# Autodesk Inventor assembly: robot
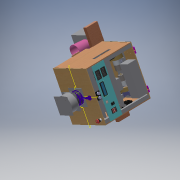
[picture p0: Inventor's stored thumbnail of the model, 180x180]
Saved by Autodesk Inventor 2019 (Build 230136000, 136)
## iProperties
Created: 2020-02-15
Part Number: robot
Document SubType Name: Assembly
Designer: franc
Author: franc
## Documents named in this file (20)
- C:\Users\franc\Desktop\EsialRobotik\Mecanique\2020\robot\robot.iam
- C:\Users\franc\Desktop\EsialRobotik\Mecanique\base_roulante\baseRoulante.iam
- C:\Users\franc\Desktop\EsialRobotik\Mecanique\2020\robot\socle-robot.ipt
- C:\Users\franc\Desktop\EsialRobotik\Mecanique\composants\Profile\calle.iam
- C:\Users\franc\Desktop\EsialRobotik\Mecanique\composants\Profile\equerreEtage.ipt
- C:\Users\franc\Desktop\EsialRobotik\Mecanique\2020\robot\profile_alu.ipt
- C:\Users\franc\Desktop\EsialRobotik\Mecanique\2020\robot\cote.ipt
- C:\Users\franc\Desktop\EsialRobotik\Mecanique\2020\robot\support-pinces.ipt
- C:\Users\franc\Desktop\EsialRobotik\Mecanique\2020\robot\pince a linge.ipt
- C:\Users\franc\Desktop\EsialRobotik\Mecanique\composants\Batterie\grosse-batterie.ipt
- C:\Users\franc\Desktop\EsialRobotik\Mecanique\composants\Batterie\petite-batterie.ipt
- C:\Users\franc\Desktop\EsialRobotik\Mecanique\2020\elements\ecueil-complet.iam
- C:\Users\franc\Desktop\EsialRobotik\Mecanique\2020\robot\étage.ipt
- C:\Users\franc\Desktop\EsialRobotik\Mecanique\2020\robot\support_arriere.iam
- C:\Users\franc\Desktop\EsialRobotik\Mecanique\2020\robot\toit.iam
- C:\Users\franc\Desktop\EsialRobotik\Mecanique\composants\AX12\AX12.iam
- C:\Users\franc\Desktop\EsialRobotik\Mecanique\composants\AX12\F3.ipt
- C:\Users\franc\Desktop\EsialRobotik\Mecanique\2020\robot\bras-manche.ipt
- C:\Users\franc\Desktop\EsialRobotik\Mecanique\2020\elements\bordure.ipt
- C:\Users\franc\Desktop\EsialRobotik\Mecanique\composants\SRF04\SRF04_sur_support.iam
## Components (48 placed, 19 different names)
1. baseRoulante:1 [sub-assembly] — Placage:1, Placage:2, Placage:3
2. socle-robot:1 — Placage:1, Placage:2, Placage:3, Placage:4, Placage:5, Placage:6, Placage:7, Placage:8, Placage:9, Placage:10, Placage:11, Placage:12, Placage:13, Placage:14, Placage:15, Placage:16, Placage:17, Placage:18, Placage:19, Placage:20, Placage:21, Placage:22, Placage:23, Placage:24, Placage:25, Placage:26, Placage:27, Placage:28, Placage:30, Placage:32, Placage:33, Placage:37, Placage:39, Placage:52, Affleurement:8, Placage:58, Placage:85
3. calle:1 [sub-assembly] — Placage:7, Placage:8, Placage:9
4. calle:2 [sub-assembly] — Placage:6, Placage:10, Placage:11
5. calle:3 [sub-assembly] — Placage:4, Placage:12, Placage:13
6. calle:4 [sub-assembly] — Placage:5, Placage:14, Placage:15, Affleurement:21
7. equerreEtage:1 — Placage:16, Placage:22, Placage:23, Placage:35, Affleurement:4
8. equerreEtage:2 — Placage:17, Placage:24, Placage:25, Placage:31, Affleurement:2
9. equerreEtage:3 — Placage:18, Placage:26, Placage:27, Placage:29, Affleurement:1
10. equerreEtage:4 — Placage:19, Placage:20, Placage:21, Placage:34, Affleurement:3
11. profile_alu:1 — Placage:28, Placage:29, Affleurement:1, Placage:59, Placage:70, Placage:74
12. profile_alu:2 — Placage:32, Placage:34, Affleurement:3, Affleurement:10, Placage:54, Placage:56, Placage:72, Placage:76, Placage:89, Affleurement:14, Placage:101, Placage:115
13. profile_alu:3 — Placage:33, Placage:35, Affleurement:4, Affleurement:5, Placage:78, Placage:82, Placage:88, Affleurement:13, Placage:107
14. profile_alu:4 — Placage:30, Placage:31, Affleurement:2, Placage:36, Placage:80, Placage:84
15. cote:1 — Placage:36, Placage:37, Affleurement:5, Affleurement:11, Placage:77, Placage:79, Placage:81, Placage:83, Placage:106
16. cote:2 — Placage:39, Affleurement:10, Placage:54, Placage:55, Placage:57, Placage:60, Placage:69, Placage:71, Placage:73, Placage:75, Placage:90, Affleurement:15, Affleurement:16, Placage:100, Placage:117, Placage:119, Affleurement:22
17. support-pinces:1 — Placage:41, Placage:42, Placage:43, Placage:44, Placage:45, Placage:47, Placage:48, Placage:49, Placage:50, Placage:51, Angle:1, Angle:2, Angle:3, Angle:4, Angle:5, Placage:55, Affleurement:11, Affleurement:22
18. pince a linge:1 — Placage:41, Placage:47, Angle:1
19. pince a linge:2 — Placage:42, Placage:48, Angle:2
20. pince a linge:3 — Placage:43, Placage:49, Angle:3
21. pince a linge:4 — Placage:44, Placage:50, Angle:4
22. pince a linge:5 — Placage:45, Placage:51, Angle:5
23. grosse-batterie:1 — Placage:52, Affleurement:8, Placage:115
24. petite-batterie:1 — Placage:116, Affleurement:18, Placage:117
25. ecueil-complet:1 [sub-assembly] — Placage:118, Affleurement:19, Affleurement:20, Placage:120
26. étage:1 — Placage:56, Placage:57, Placage:58, Placage:61, Placage:62, Placage:63, Placage:64, Placage:99, Placage:105, Placage:116, Affleurement:18
27. étage:2 — Placage:59, Placage:60, Placage:65, Placage:66, Placage:67, Placage:68, Placage:85
28. equerreEtage:5 — Placage:64, Placage:83, Placage:84
29. equerreEtage:6 — Placage:63, Placage:81, Placage:82
30. equerreEtage:7 — Placage:61, Placage:69, Placage:70
31. equerreEtage:8 — Placage:62, Placage:71, Placage:72
32. equerreEtage:9 — Placage:68, Placage:77, Placage:78
33. equerreEtage:10 — Placage:65, Placage:73, Placage:74
34. equerreEtage:11 — Placage:67, Placage:79, Placage:80
35. equerreEtage:12 — Placage:66, Placage:75, Placage:76
36. support_arriere:1 [sub-assembly] — Placage:88, Placage:89, Affleurement:13, Affleurement:14
37. toit:1 [sub-assembly] — Placage:90, Affleurement:15, Affleurement:16, Placage:120, Placage:121, Placage:122, Placage:123, Placage:124, Placage:125, Placage:126, Placage:127, Placage:128
38. AX12:1 [sub-assembly] — Placage:96, Placage:97, Placage:98, Placage:100, Placage:111, Placage:112, Placage:113
39. AX12:2 [sub-assembly] — Placage:102, Placage:103, Placage:104, Placage:106, Placage:108, Placage:109, Placage:110
40. F3:1 — Placage:96, Placage:97, Placage:98, Placage:99, Placage:101
41. F3:2 — Placage:102, Placage:103, Placage:104, Placage:105, Placage:107
42. bras-manche:1 — Placage:108, Placage:109, Placage:110
43. bras-manche:2 — Placage:111, Placage:112, Placage:113
44. bordure:1 — Placage:118, Affleurement:19, Affleurement:20, Affleurement:21, Placage:119
45. SRF04_sur_support:1 [sub-assembly] — Placage:125, Placage:126
46. SRF04_sur_support:2 [sub-assembly] — Placage:127, Placage:128
47. SRF04_sur_support:3 [sub-assembly] — Placage:121, Placage:122
48. SRF04_sur_support:4 [sub-assembly] — Placage:123, Placage:124
## Relationships (138: Mate 116, Flush 17, Angle 5)
- Placage:1 [Mate]: baseRoulante:1 ↔ socle-robot:1
- Placage:2 [Mate]: baseRoulante:1 ↔ socle-robot:1
- Placage:3 [Mate]: baseRoulante:1 ↔ socle-robot:1
- Placage:4 [Mate]: socle-robot:1 ↔ calle:3
- Placage:5 [Mate]: socle-robot:1 ↔ calle:4
- Placage:6 [Mate]: socle-robot:1 ↔ calle:2
- Placage:7 [Mate]: socle-robot:1 ↔ calle:1
- Placage:8 [Mate]: socle-robot:1 ↔ calle:1
- Placage:9 [Mate]: socle-robot:1 ↔ calle:1
- Placage:10 [Mate]: socle-robot:1 ↔ calle:2
- Placage:11 [Mate]: socle-robot:1 ↔ calle:2
- Placage:12 [Mate]: socle-robot:1 ↔ calle:3
- Placage:13 [Mate]: socle-robot:1 ↔ calle:3
- Placage:14 [Mate]: socle-robot:1 ↔ calle:4
- Placage:15 [Mate]: socle-robot:1 ↔ calle:4
- Placage:16 [Mate]: socle-robot:1 ↔ equerreEtage:1
- Placage:17 [Mate]: socle-robot:1 ↔ equerreEtage:2
- Placage:18 [Mate]: socle-robot:1 ↔ equerreEtage:3
- Placage:19 [Mate]: socle-robot:1 ↔ equerreEtage:4
- Placage:20 [Mate]: socle-robot:1 ↔ equerreEtage:4
- Placage:21 [Mate]: socle-robot:1 ↔ equerreEtage:4
- Placage:22 [Mate]: socle-robot:1 ↔ equerreEtage:1
- Placage:23 [Mate]: socle-robot:1 ↔ equerreEtage:1
- Placage:24 [Mate]: socle-robot:1 ↔ equerreEtage:2
- Placage:25 [Mate]: socle-robot:1 ↔ equerreEtage:2
- Placage:26 [Mate]: socle-robot:1 ↔ equerreEtage:3
- Placage:27 [Mate]: socle-robot:1 ↔ equerreEtage:3
- Placage:28 [Mate]: socle-robot:1 ↔ profile_alu:1
- Placage:29 [Mate]: equerreEtage:3 ↔ profile_alu:1
- Affleurement:1 [Flush]: equerreEtage:3 ↔ profile_alu:1
- Placage:30 [Mate]: socle-robot:1 ↔ profile_alu:4
- Placage:31 [Mate]: equerreEtage:2 ↔ profile_alu:4
- Affleurement:2 [Flush]: equerreEtage:2 ↔ profile_alu:4
- Placage:32 [Mate]: socle-robot:1 ↔ profile_alu:2
- Placage:33 [Mate]: socle-robot:1 ↔ profile_alu:3
- Placage:34 [Mate]: equerreEtage:4 ↔ profile_alu:2
- Affleurement:3 [Flush]: equerreEtage:4 ↔ profile_alu:2
- Placage:35 [Mate]: equerreEtage:1 ↔ profile_alu:3
- Affleurement:4 [Flush]: equerreEtage:1 ↔ profile_alu:3
- Placage:36 [Mate]: profile_alu:4 ↔ cote:1
- Placage:37 [Mate]: socle-robot:1 ↔ cote:1
- Affleurement:5 [Flush]: profile_alu:3 ↔ cote:1
- Placage:39 [Mate]: socle-robot:1 ↔ cote:2
- Placage:41 [Mate]: support-pinces:1 ↔ pince a linge:1
- Placage:42 [Mate]: support-pinces:1 ↔ pince a linge:2
- Placage:43 [Mate]: support-pinces:1 ↔ pince a linge:3
- Placage:44 [Mate]: support-pinces:1 ↔ pince a linge:4
- Placage:45 [Mate]: support-pinces:1 ↔ pince a linge:5
- Placage:47 [Mate]: support-pinces:1 ↔ pince a linge:1
- Placage:48 [Mate]: support-pinces:1 ↔ pince a linge:2
- Placage:49 [Mate]: support-pinces:1 ↔ pince a linge:3
- Placage:50 [Mate]: support-pinces:1 ↔ pince a linge:4
- Placage:51 [Mate]: support-pinces:1 ↔ pince a linge:5
- Angle:1 (0 deg): support-pinces:1 ↔ pince a linge:1
- Angle:2 (0 deg): support-pinces:1 ↔ pince a linge:2
- Angle:3 (0 deg): support-pinces:1 ↔ pince a linge:3
- Angle:4 (0 deg): support-pinces:1 ↔ pince a linge:4
- Angle:5 (0 deg): support-pinces:1 ↔ pince a linge:5
- Placage:52 [Mate]: socle-robot:1 ↔ grosse-batterie:1
- Affleurement:8 [Flush]: socle-robot:1 ↔ grosse-batterie:1
- Affleurement:10 [Flush]: profile_alu:2 ↔ cote:2
- Placage:54 [Mate]: profile_alu:2 ↔ cote:2
- Placage:55 [Mate]: cote:2 ↔ support-pinces:1
- Affleurement:11 [Flush] (-5 mm): cote:1 ↔ support-pinces:1
- Placage:56 [Mate]: profile_alu:2 ↔ étage:1
- Placage:57 [Mate]: cote:2 ↔ étage:1
- Placage:58 [Mate] (140 mm): socle-robot:1 ↔ étage:1
- Placage:59 [Mate]: profile_alu:1 ↔ étage:2
- Placage:60 [Mate]: cote:2 ↔ étage:2
- Placage:61 [Mate]: étage:1 ↔ equerreEtage:7
- Placage:62 [Mate]: étage:1 ↔ equerreEtage:8
- Placage:63 [Mate]: étage:1 ↔ equerreEtage:6
- Placage:64 [Mate]: étage:1 ↔ equerreEtage:5
- Placage:65 [Mate]: étage:2 ↔ equerreEtage:10
- Placage:66 [Mate]: étage:2 ↔ equerreEtage:12
- Placage:67 [Mate]: étage:2 ↔ equerreEtage:11
- Placage:68 [Mate]: étage:2 ↔ equerreEtage:9
- Placage:69 [Mate]: cote:2 ↔ equerreEtage:7
- Placage:70 [Mate]: profile_alu:1 ↔ equerreEtage:7
- Placage:71 [Mate]: cote:2 ↔ equerreEtage:8
- Placage:72 [Mate]: profile_alu:2 ↔ equerreEtage:8
- Placage:73 [Mate]: cote:2 ↔ equerreEtage:10
- Placage:74 [Mate]: profile_alu:1 ↔ equerreEtage:10
- Placage:75 [Mate]: cote:2 ↔ equerreEtage:12
- Placage:76 [Mate]: profile_alu:2 ↔ equerreEtage:12
- Placage:77 [Mate]: cote:1 ↔ equerreEtage:9
- Placage:78 [Mate]: profile_alu:3 ↔ equerreEtage:9
- Placage:79 [Mate]: cote:1 ↔ equerreEtage:11
- Placage:80 [Mate]: profile_alu:4 ↔ equerreEtage:11
- Placage:81 [Mate]: cote:1 ↔ equerreEtage:6
- Placage:82 [Mate]: profile_alu:3 ↔ equerreEtage:6
- Placage:83 [Mate]: cote:1 ↔ equerreEtage:5
- Placage:84 [Mate]: profile_alu:4 ↔ equerreEtage:5
- Placage:85 [Mate] (230 mm): socle-robot:1 ↔ étage:2
- Placage:88 [Mate]: profile_alu:3 ↔ support_arriere:1
- Placage:89 [Mate]: profile_alu:2 ↔ support_arriere:1
- Affleurement:13 [Flush] (30 mm): profile_alu:3 ↔ support_arriere:1
- Affleurement:14 [Flush]: profile_alu:2 ↔ support_arriere:1
- Placage:90 [Mate]: cote:2 ↔ toit:1
- Affleurement:15 [Flush]: cote:2 ↔ toit:1
- Affleurement:16 [Flush]: cote:2 ↔ toit:1
- Placage:96 [Mate]: AX12:1 ↔ F3:1
- Placage:97 [Mate]: AX12:1 ↔ F3:1
- Placage:98 [Mate]: AX12:1 ↔ F3:1
- Placage:99 [Mate]: étage:1 ↔ F3:1
- Placage:100 [Mate]: cote:2 ↔ AX12:1
- Placage:101 [Mate]: profile_alu:2 ↔ F3:1
- Placage:102 [Mate]: AX12:2 ↔ F3:2
- Placage:103 [Mate]: AX12:2 ↔ F3:2
- Placage:104 [Mate]: AX12:2 ↔ F3:2
- Placage:105 [Mate]: étage:1 ↔ F3:2
- Placage:106 [Mate]: cote:1 ↔ AX12:2
- Placage:107 [Mate]: profile_alu:3 ↔ F3:2
- Placage:108 [Mate]: AX12:2 ↔ bras-manche:1
- Placage:109 [Mate]: AX12:2 ↔ bras-manche:1
- Placage:110 [Mate]: AX12:2 ↔ bras-manche:1
- Placage:111 [Mate]: AX12:1 ↔ bras-manche:2
- Placage:112 [Mate]: AX12:1 ↔ bras-manche:2
- Placage:113 [Mate]: AX12:1 ↔ bras-manche:2
- Placage:115 [Mate] (5 mm): profile_alu:2 ↔ grosse-batterie:1
- Placage:116 [Mate]: petite-batterie:1 ↔ étage:1
- Affleurement:18 [Flush]: petite-batterie:1 ↔ étage:1
- Placage:117 [Mate] (100 mm): cote:2 ↔ petite-batterie:1
- Placage:118 [Mate]: ecueil-complet:1 ↔ bordure:1
- Affleurement:19 [Flush]: ecueil-complet:1 ↔ bordure:1
- Affleurement:20 [Flush] (-40.5 mm): ecueil-complet:1 ↔ bordure:1
- Affleurement:21 [Flush]: calle:4 ↔ bordure:1
- Placage:119 [Mate]: cote:2 ↔ bordure:1
- Affleurement:22 [Flush] (45 mm): cote:2 ↔ support-pinces:1
- Placage:120 [Mate]: ecueil-complet:1 ↔ toit:1
- Placage:121 [Mate]: toit:1 ↔ SRF04_sur_support:3
- Placage:122 [Mate]: toit:1 ↔ SRF04_sur_support:3
- Placage:123 [Mate]: toit:1 ↔ SRF04_sur_support:4
- Placage:124 [Mate]: toit:1 ↔ SRF04_sur_support:4
- Placage:125 [Mate]: toit:1 ↔ SRF04_sur_support:1
- Placage:126 [Mate]: toit:1 ↔ SRF04_sur_support:1
- Placage:127 [Mate]: toit:1 ↔ SRF04_sur_support:2
- Placage:128 [Mate]: toit:1 ↔ SRF04_sur_support:2
